# Autodesk Inventor assembly: shoot
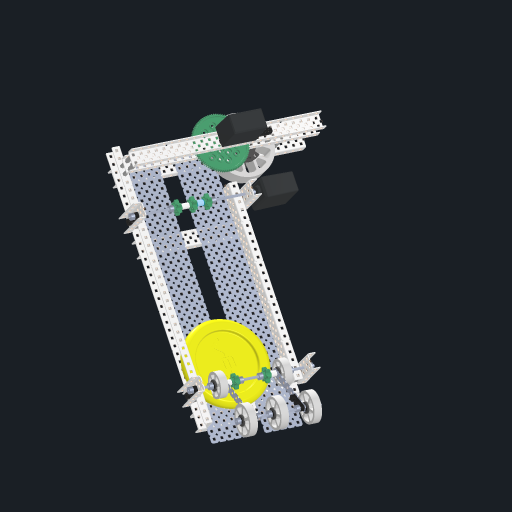
[picture p0: Inventor's stored thumbnail of the model, 512x512]
Saved by Autodesk Inventor 2023 (Build 270158000, 158)
## iProperties
Created: 2023-03-08
Part Number: shoot
Document SubType Name: Assembly
Designer: Windows Macbook
Author: Windows Macbook
## Documents named in this file (39)
- C:\Users\Windows Macbook\Desktop\VRC-SPIN-UP\Inventor\Assembly\Pre Worlds\V1\shoot.iam
- C:\Users\Windows Macbook\Desktop\VRC-SPIN-UP\Inventor\Structure\C Channel\Aluminum 1x2x1\Alu C 1x2x1x35.ipt
- C:\Users\Windows Macbook\Desktop\VRC-SPIN-UP\Inventor\Structure\C Channel\Aluminum 1x2x1\Alu C 1x2x1x14.ipt
- C:\Users\Windows Macbook\Desktop\VRC-SPIN-UP\Inventor\Structure\Plate\Steel\Steel Plate 5x25.ipt
- C:\Users\Windows Macbook\Desktop\VRC-SPIN-UP\Inventor\Structure\Plate\Steel\Steel Plate 5x10.ipt
- C:\Users\Windows Macbook\Desktop\VRC-SPIN-UP\Inventor\Structure\C Channel\Aluminum 1x2x1\Alu C 1x2x1x25.ipt
- C:\Users\Windows Macbook\Desktop\VRC-SPIN-UP\Inventor\Motion\Wheels\Flex Wheels\4 Flex, LS.iam
- C:\Users\Windows Macbook\Desktop\VRC-SPIN-UP\Inventor\Structure\Standoff\Standoff .50.ipt
- C:\Users\Windows Macbook\Desktop\VRC-SPIN-UP\Inventor\Structure\Standoff.ipt
- C:\Users\Windows Macbook\Desktop\VRC-SPIN-UP\Inventor\Structure\C Channel\Aluminum 1x3x1\Alu C 1x3x1x14.ipt
- C:\Users\Windows Macbook\Desktop\VRC-SPIN-UP\Inventor\Motion\Spacers\Spacer Nylon .375 OD\NSpacer .375 OD x .500.ipt
- C:\Users\Windows Macbook\Desktop\VRC-SPIN-UP\Inventor\Motion\Spacers\Spacer Nylon .375 OD.ipt
- C:\Users\Windows Macbook\Desktop\VRC-SPIN-UP\Inventor\Motion\Spacers\Spacer Nylon .375 OD\NSpacer .375 OD x .250.ipt
- C:\Users\Windows Macbook\Desktop\VRC-SPIN-UP\Inventor\Structure\Hardware\Screw Steel - Star.ipt
- C:\Users\Windows Macbook\Desktop\VRC-SPIN-UP\Inventor\Structure\Hardware\Screw Steel - Star\SScrew Star Smooth 1.000.ipt
- C:\Users\Windows Macbook\Desktop\VRC-SPIN-UP\Inventor\Structure\Hardware\Nut Nylock.ipt
- C:\Users\Windows Macbook\Desktop\VRC-SPIN-UP\Inventor\Motion\Shaft LS\Bearing Flat.ipt
- C:\Users\Windows Macbook\Desktop\VRC-SPIN-UP\Inventor\Motion\Spacers\Spacer Nylon .313 OD.ipt
- C:\Users\Windows Macbook\Desktop\VRC-SPIN-UP\Inventor\Motion\Gears\HS Gear\HS 12T Gear, Square.iam
- C:\Users\Windows Macbook\Desktop\VRC-SPIN-UP\Inventor\Motion\Gears\HS Gear.iam
- C:\Users\Windows Macbook\Desktop\VRC-SPIN-UP\Inventor\Motion\Gears\LS 84T Gear.ipt
- C:\Users\Windows Macbook\Desktop\VRC-SPIN-UP\Inventor\Motion\Spacers\Spacer Nylon .313 OD\NSpacer .313 OD x .125.ipt
- C:\Users\Windows Macbook\Desktop\VRC-SPIN-UP\Inventor\Motion\Spacers\Spacer Nylon .313 OD\NSpacer .313 OD x .250.ipt
- C:\Users\Windows Macbook\Desktop\VRC-SPIN-UP\Inventor\Structure\Standoff\Standoff 1.00.ipt
- C:\Users\Windows Macbook\Desktop\VRC-SPIN-UP\Inventor\Structure\Plate\Steel\Steel Plate 1x8.ipt
- C:\Users\Windows Macbook\Desktop\VRC-SPIN-UP\Inventor\Disk.ipt
- C:\Users\Windows Macbook\Desktop\VRC-SPIN-UP\Inventor\Structure\C Channel\Aluminum 1x2x1\Alu C 1x2x1x5.ipt
- C:\Users\Windows Macbook\Desktop\VRC-SPIN-UP\Inventor\Motion\Shaft LS\Shaft LS\Shaft LS 8.0.ipt
- C:\Users\Windows Macbook\Desktop\VRC-SPIN-UP\Inventor\Motion\Shaft LS\Shaft LS.ipt
- C:\Users\Windows Macbook\Desktop\VRC-SPIN-UP\Inventor\Motion\Wheels\Flex Wheels\1.625 Flex, LS.iam
- C:\Users\Windows Macbook\Desktop\VRC-SPIN-UP\Inventor\Motion\Reference Files\Shaft Collar Metal.ipt
- C:\Users\Windows Macbook\Desktop\VRC-SPIN-UP\Inventor\Motion\Wheels\Flex Wheels\2 Flex, LS.iam
- C:\Users\Windows Macbook\Desktop\VRC-SPIN-UP\Inventor\Motion\Shaft LS\Shaft LS\Shaft LS 5.5.ipt
- C:\Users\Windows Macbook\Desktop\VRC-SPIN-UP\Inventor\Motion\Sprockets\9P Sprocket.iam
- C:\Users\Windows Macbook\Desktop\VRC-SPIN-UP\Inventor\Motion\Spacers\Spacer Nylon .313 OD\NSpacer .313 OD x .375.ipt
- C:\Users\Windows Macbook\Desktop\VRC-SPIN-UP\Inventor\Motion\Sprockets\9P Sprocket\9P 6T Sprocket, Square.iam
- C:\Users\Windows Macbook\Desktop\VRC-SPIN-UP\Inventor\Electronics\V5 Simple Motor.ipt
- C:\Users\Windows Macbook\Desktop\VRC-SPIN-UP\Inventor\Structure\Standoff\Standoff .75.ipt
- C:\Users\Windows Macbook\Desktop\VRC-SPIN-UP\Inventor\Motion\Spacers\Spacer Nylon .313 OD\NSpacer .313 OD x .500.ipt
## Components (97 placed, 31 different names)
1. Alu C 1x2x1x35:1 — Insert:1, Insert:2, Insert:15, Insert:16, Insert:18, Insert:19, Insert:22, Insert:23, Insert:43, Insert:44, Insert:91, Insert:92
2. Alu C 1x2x1x25:1 — Insert:17, Insert:117, Insert:118, Insert:119, Insert:120
3. Alu C 1x2x1x14:2 — Insert:1, Insert:2, Insert:7, Insert:8, Insert:9, Insert:10, Insert:24, Insert:26
4. Alu C 1x2x1x25:3 — Insert:5, Insert:6, Insert:69, Insert:70, Angle:1, Insert:96, Insert:97
5. Steel Plate 5x25:1 — Insert:9, Insert:10, Mate:1
6. Steel Plate 5x25:2 — Insert:7, Insert:8
7. Steel Plate 5x10:1
8. Steel Plate 5x10:2
9. Alu C 1x2x1x14:3 — Insert:15, Insert:16
10. 4 Flex, LS:1 [sub-assembly] — Insert:17, Insert:114
11. Standoff .75:1 — Insert:19, Insert:21
12. Standoff .75:2 — Insert:18, Insert:20
13. Alu C 1x2x1x25:2 — Insert:20, Insert:21, Insert:28, Insert:29, Insert:32, Insert:33, Insert:37, Insert:38, Insert:123, Insert:124
14. Alu C 1x3x1x14:1 — Insert:22, Insert:23, Insert:5, Insert:6
15. NSpacer .375 OD x .500:1 — Insert:24, Insert:25
16. NSpacer .375 OD x .250:2 — Insert:25, Insert:27
17. SScrew Star Smooth 1.000:1 — Insert:26
18. Nut Nylock:1 — Insert:27
19. Bearing Flat:1 — Insert:28, Insert:29, Insert:30
20. NSpacer .313 OD x .250:1 — Insert:30, Insert:31
21. HS 12T Gear, Square:1 [sub-assembly] — Insert:31
22. LS 84T Gear:1 — Insert:34, Insert:36
23. Bearing Flat:2 — Insert:32, Insert:33, Insert:35
24. NSpacer .313 OD x .125:2 — Insert:34, Insert:35
25. NSpacer .313 OD x .125:3 — Insert:36
26. Standoff 1.00:3 — Insert:38
27. Standoff 1.00:4 — Insert:37
28. Alu C 1x2x1x25:4 — Insert:121, Insert:122, Insert:125, Insert:126, Insert:128, Insert:129
29. Steel Plate 1x8:1 — Insert:52, Insert:53, Insert:54, Insert:56, Insert:78
30. Alu C 1x2x1x5:2 — Insert:45, Insert:46, Insert:47, Insert:48, Insert:49
31. Standoff .50:7 — Insert:44, Insert:46
32. Standoff .50:8 — Insert:43, Insert:45
33. Disk:2 — Mate:1
34. Bearing Flat:3 — Insert:47, Insert:48, Flush:1, Cylindrical:1, Insert:104
35. Shaft LS 8.0:1 — Flush:1, Cylindrical:1
36. 1.625 Flex, LS:1 [sub-assembly] — Insert:49, Insert:50, Insert:56
37. Shaft Collar Metal:1 — Insert:50
38. 2 Flex, LS:1 [sub-assembly] — Insert:52, Insert:58
39. Shaft Collar Metal:2 — Insert:55, Insert:76
40. Bearing Flat:4 — Insert:53, Insert:54, Insert:55
41. NSpacer .313 OD x .375:5 — Insert:78, Insert:79
42. Shaft Collar Metal:4 — Insert:58, Flush:2, Cylindrical:2
43. Steel Plate 1x8:2 — Insert:77
44. 1.625 Flex, LS:2 [sub-assembly] — Insert:72, Insert:73
45. 2 Flex, LS:2 [sub-assembly] — Insert:66
46. Shaft Collar Metal:6
47. Bearing Flat:5
48. NSpacer .313 OD x .375:4 — Insert:77, Insert:80
49. Shaft Collar Metal:8 — Insert:66, Cylindrical:3
50. Alu C 1x2x1x5:3 — Insert:71, Angle:1, Insert:72
51. Bearing Flat:6 — Insert:103
52. Standoff .50:9 — Insert:69
53. Standoff .50:10 — Insert:70, Insert:71
54. Shaft Collar Metal:9 — Insert:73
55. Shaft LS 5.5:2 — Flush:2, Cylindrical:2, Cylindrical:3
56. 2 Flex, LS:3 [sub-assembly] — Insert:74, Insert:75
57. Shaft Collar Metal:10 — Insert:75
58. Shaft Collar Metal:11 — Insert:74, Insert:76
59. 9P 6T Sprocket, Square:1 [sub-assembly] — Insert:79, Insert:82
60. 9P 6T Sprocket, Square:2 [sub-assembly] — Insert:80, Insert:81
61. Shaft Collar Metal:12 — Insert:82
62. Shaft Collar Metal:13 — Insert:81
63. Alu C 1x2x1x5:4 — Insert:95
64. Standoff .50:11 — Insert:92
65. Standoff .50:12 — Insert:91
66. Bearing Flat:7 — Insert:101
67. Shaft LS 8.0:3
68. Alu C 1x2x1x5:5 — Insert:90, Insert:100
69. Bearing Flat:8 — Insert:105, Insert:106, Insert:110
70. Standoff .50:13 — Insert:90, Insert:97
71. Standoff .50:14 — Insert:96
72. 9P 6T Sprocket, Square:3 [sub-assembly] — Insert:94, Insert:139
73. Shaft Collar Metal:15 — Insert:94, Insert:95
74. 9P 6T Sprocket, Square:4 [sub-assembly] — Insert:140
75. Shaft Collar Metal:16 — Insert:100
76. Shaft Collar Metal:19 — Insert:103
77. Shaft Collar Metal:20 — Insert:101
78. Shaft Collar Metal:21 — Insert:104
79. V5 Simple Motor:1 — Insert:105, Insert:106
80. V5 Simple Motor:2 — Insert:130, Insert:131
81. Shaft Collar Metal:23 — Insert:110
82. Shaft Collar Metal:24 — Insert:113
83. Shaft Collar Metal:26 — Insert:111
84. NSpacer .313 OD x .250:6 — Insert:114
85. Standoff 1.00:15 — Insert:115
86. Standoff .75:16 — Insert:115, Insert:118
87. Standoff 1.00:17
88. Standoff .75:18 — Insert:117
89. Bearing Flat:9 — Insert:119, Insert:120, Insert:113
90. Bearing Flat:10 — Insert:121, Insert:111, Insert:122, Insert:130, Insert:131
91. Standoff 1.00:19 — Insert:123, Insert:126
92. Standoff 1.00:20 — Insert:124, Insert:125
93. Shaft Collar Metal:27
94. Bearing Flat:11 — Insert:128, Insert:129
95. 9P 6T Sprocket, Square:5 [sub-assembly] — Insert:141
96. NSpacer .313 OD x .500:8 — Insert:139, Insert:141
97. NSpacer .313 OD x .500:9 — Insert:140
## Relationships (128: Insert 119, CylindricalJoint 4, Flush 3, Mate 1, Angle 1)
- Insert:1: Alu C 1x2x1x35:1 ↔ Alu C 1x2x1x14:2
- Insert:2: Alu C 1x2x1x35:1 ↔ Alu C 1x2x1x14:2
- [Insert]: Alu C 1x2x1x35:1 ↔ Alu C 1x2x1x25:1
- [Insert]: Alu C 1x2x1x35:1 ↔ Alu C 1x2x1x25:1
- Insert:5: Alu C 1x2x1x25:3 ↔ Alu C 1x3x1x14:1
- Insert:6: Alu C 1x2x1x25:3 ↔ Alu C 1x3x1x14:1
- Insert:7: Alu C 1x2x1x14:2 ↔ Steel Plate 5x25:2
- Insert:8: Alu C 1x2x1x14:2 ↔ Steel Plate 5x25:2
- Insert:9: Alu C 1x2x1x14:2 ↔ Steel Plate 5x25:1
- Insert:10: Alu C 1x2x1x14:2 ↔ Steel Plate 5x25:1
- [Insert]: Alu C 1x2x1x25:1 ↔ Steel Plate 5x10:1
- [Insert]: Alu C 1x2x1x25:1 ↔ Steel Plate 5x10:1
- [Insert]: Alu C 1x2x1x25:1 ↔ Steel Plate 5x10:2
- [Insert]: Alu C 1x2x1x25:1 ↔ Steel Plate 5x10:2
- Insert:15: Alu C 1x2x1x35:1 ↔ Alu C 1x2x1x14:3
- Insert:16: Alu C 1x2x1x35:1 ↔ Alu C 1x2x1x14:3
- Insert:17: Alu C 1x2x1x25:1 ↔ 4 Flex, LS:1
- Insert:18: Alu C 1x2x1x35:1 ↔ Standoff .75:2
- Insert:19: Alu C 1x2x1x35:1 ↔ Standoff .75:1
- Insert:20: Standoff .75:2 ↔ Alu C 1x2x1x25:2
- Insert:21: Standoff .75:1 ↔ Alu C 1x2x1x25:2
- Insert:22: Alu C 1x2x1x35:1 ↔ Alu C 1x3x1x14:1
- Insert:23: Alu C 1x2x1x35:1 ↔ Alu C 1x3x1x14:1
- Insert:24: Alu C 1x2x1x14:2 ↔ NSpacer .375 OD x .500:1
- Insert:25: NSpacer .375 OD x .500:1 ↔ NSpacer .375 OD x .250:2
- Insert:26: Alu C 1x2x1x14:2 ↔ SScrew Star Smooth 1.000:1
- Insert:27: NSpacer .375 OD x .250:2 ↔ Nut Nylock:1
- Insert:28: Alu C 1x2x1x25:2 ↔ Bearing Flat:1
- Insert:29: Alu C 1x2x1x25:2 ↔ Bearing Flat:1
- Insert:30: Bearing Flat:1 ↔ NSpacer .313 OD x .250:1
- Insert:31: NSpacer .313 OD x .250:1 ↔ HS 12T Gear, Square:1
- Insert:32: Alu C 1x2x1x25:2 ↔ Bearing Flat:2
- Insert:33: Alu C 1x2x1x25:2 ↔ Bearing Flat:2
- Insert:34: LS 84T Gear:1 ↔ NSpacer .313 OD x .125:2
- Insert:35: Bearing Flat:2 ↔ NSpacer .313 OD x .125:2
- Insert:36: LS 84T Gear:1 ↔ NSpacer .313 OD x .125:3
- Insert:37: Alu C 1x2x1x25:2 ↔ Standoff 1.00:4
- Insert:38: Alu C 1x2x1x25:2 ↔ Standoff 1.00:3
- Insert:43: Alu C 1x2x1x35:1 ↔ Standoff .50:8
- Insert:44: Alu C 1x2x1x35:1 ↔ Standoff .50:7
- Insert:45: Alu C 1x2x1x5:2 ↔ Standoff .50:8
- Insert:46: Alu C 1x2x1x5:2 ↔ Standoff .50:7
- Mate:1: Steel Plate 5x25:1 ↔ Disk:2
- Insert:47: Alu C 1x2x1x5:2 ↔ Bearing Flat:3
- Insert:48: Alu C 1x2x1x5:2 ↔ Bearing Flat:3
- Flush:1: Bearing Flat:3 ↔ Shaft LS 8.0:1
- Cylindrical:1: Bearing Flat:3 ↔ Shaft LS 8.0:1
- Insert:49 (25.4 mm): Alu C 1x2x1x5:2 ↔ 1.625 Flex, LS:1
- Insert:50: 1.625 Flex, LS:1 ↔ Shaft Collar Metal:1
- Insert:52: Steel Plate 1x8:1 ↔ 2 Flex, LS:1
- Insert:53: Steel Plate 1x8:1 ↔ Bearing Flat:4
- Insert:54: Steel Plate 1x8:1 ↔ Bearing Flat:4
- Insert:55: Shaft Collar Metal:2 ↔ Bearing Flat:4
- Insert:56: Steel Plate 1x8:1 ↔ 1.625 Flex, LS:1
- Insert:58: 2 Flex, LS:1 ↔ Shaft Collar Metal:4
- [Insert]: Steel Plate 1x8:2 ↔ 2 Flex, LS:2
- [Insert]: Steel Plate 1x8:2 ↔ Bearing Flat:5
- [Insert]: Steel Plate 1x8:2 ↔ Bearing Flat:5
- [Insert]: Shaft Collar Metal:6 ↔ Bearing Flat:5
- [Insert]: Steel Plate 1x8:2 ↔ 1.625 Flex, LS:2
- Insert:66: 2 Flex, LS:2 ↔ Shaft Collar Metal:8
- [Insert]: Alu C 1x2x1x5:3 ↔ Bearing Flat:6
- [Insert]: Alu C 1x2x1x5:3 ↔ Bearing Flat:6
- Insert:69: Alu C 1x2x1x25:3 ↔ Standoff .50:9
- Insert:70: Alu C 1x2x1x25:3 ↔ Standoff .50:10
- Insert:71: Alu C 1x2x1x5:3 ↔ Standoff .50:10
- Angle:1 (0 deg): Alu C 1x2x1x25:3 ↔ Alu C 1x2x1x5:3
- Insert:72 (25.4 mm): 1.625 Flex, LS:2 ↔ Alu C 1x2x1x5:3
- Insert:73: 1.625 Flex, LS:2 ↔ Shaft Collar Metal:9
- Flush:2: Shaft Collar Metal:4 ↔ Shaft LS 5.5:2
- Cylindrical:2: Shaft Collar Metal:4 ↔ Shaft LS 5.5:2
- Cylindrical:3: Shaft Collar Metal:8 ↔ Shaft LS 5.5:2
- Insert:74: 2 Flex, LS:3 ↔ Shaft Collar Metal:11
- Insert:75: 2 Flex, LS:3 ↔ Shaft Collar Metal:10
- Insert:76 (12.7 mm): Shaft Collar Metal:2 ↔ Shaft Collar Metal:11
- Insert:77: Steel Plate 1x8:2 ↔ NSpacer .313 OD x .375:4
- Insert:78: Steel Plate 1x8:1 ↔ NSpacer .313 OD x .375:5
- Insert:79: NSpacer .313 OD x .375:5 ↔ 9P 6T Sprocket, Square:1
- Insert:80: NSpacer .313 OD x .375:4 ↔ 9P 6T Sprocket, Square:2
- Insert:81: 9P 6T Sprocket, Square:2 ↔ Shaft Collar Metal:13
- Insert:82: 9P 6T Sprocket, Square:1 ↔ Shaft Collar Metal:12
- [Insert]: Alu C 1x2x1x5:4 ↔ Standoff .50:12
- [Insert]: Alu C 1x2x1x5:4 ↔ Standoff .50:11
- [Insert]: Alu C 1x2x1x5:4 ↔ Bearing Flat:7
- [Insert]: Alu C 1x2x1x5:4 ↔ Bearing Flat:7
- [Flush]: Bearing Flat:7 ↔ Shaft LS 8.0:3
- [CylindricalJoint]: Bearing Flat:7 ↔ Shaft LS 8.0:3
- [Insert]: Alu C 1x2x1x5:5 ↔ Bearing Flat:8
- [Insert]: Alu C 1x2x1x5:5 ↔ Bearing Flat:8
- [Insert]: Alu C 1x2x1x5:5 ↔ Standoff .50:14
- Insert:90: Alu C 1x2x1x5:5 ↔ Standoff .50:13
- Insert:91: Alu C 1x2x1x35:1 ↔ Standoff .50:12
- Insert:92: Alu C 1x2x1x35:1 ↔ Standoff .50:11
- Insert:94: 9P 6T Sprocket, Square:3 ↔ Shaft Collar Metal:15
- Insert:95 (50.8 mm): Alu C 1x2x1x5:4 ↔ Shaft Collar Metal:15
- Insert:96: Alu C 1x2x1x25:3 ↔ Standoff .50:14
- Insert:97: Alu C 1x2x1x25:3 ↔ Standoff .50:13
- [Insert]: 9P 6T Sprocket, Square:4 ↔ Shaft Collar Metal:16
- Insert:100 (50.8 mm): Alu C 1x2x1x5:5 ↔ Shaft Collar Metal:16
- Insert:101: Bearing Flat:7 ↔ Shaft Collar Metal:20
- Insert:103: Bearing Flat:6 ↔ Shaft Collar Metal:19
- Insert:104: Bearing Flat:3 ↔ Shaft Collar Metal:21
- Insert:105: Bearing Flat:8 ↔ V5 Simple Motor:1
- Insert:106: Bearing Flat:8 ↔ V5 Simple Motor:1
- Insert:110: Bearing Flat:8 ↔ Shaft Collar Metal:23
- Insert:111: Shaft Collar Metal:26 ↔ Bearing Flat:10
- Insert:113: Shaft Collar Metal:24 ↔ Bearing Flat:9
- Insert:114: 4 Flex, LS:1 ↔ NSpacer .313 OD x .250:6
- Insert:115: Standoff 1.00:15 ↔ Standoff .75:16
- [Insert]: Standoff 1.00:17 ↔ Standoff .75:18
- Insert:117: Alu C 1x2x1x25:1 ↔ Standoff .75:18
- Insert:118: Alu C 1x2x1x25:1 ↔ Standoff .75:16
- Insert:119: Alu C 1x2x1x25:1 ↔ Bearing Flat:9
- Insert:120: Alu C 1x2x1x25:1 ↔ Bearing Flat:9
- Insert:121: Alu C 1x2x1x25:4 ↔ Bearing Flat:10
- Insert:122: Alu C 1x2x1x25:4 ↔ Bearing Flat:10
- Insert:123: Alu C 1x2x1x25:2 ↔ Standoff 1.00:19
- Insert:124: Alu C 1x2x1x25:2 ↔ Standoff 1.00:20
- Insert:125: Alu C 1x2x1x25:4 ↔ Standoff 1.00:20
- Insert:126: Alu C 1x2x1x25:4 ↔ Standoff 1.00:19
- [Insert]: Shaft Collar Metal:27 ↔ Bearing Flat:11
- Insert:128: Alu C 1x2x1x25:4 ↔ Bearing Flat:11
- Insert:129: Alu C 1x2x1x25:4 ↔ Bearing Flat:11
- Insert:130: V5 Simple Motor:2 ↔ Bearing Flat:10
- Insert:131: V5 Simple Motor:2 ↔ Bearing Flat:10
- Insert:139: 9P 6T Sprocket, Square:3 ↔ NSpacer .313 OD x .500:8
- Insert:140: 9P 6T Sprocket, Square:4 ↔ NSpacer .313 OD x .500:9
- Insert:141: 9P 6T Sprocket, Square:5 ↔ NSpacer .313 OD x .500:8
## Named parameters: d65_d57 = 0 mm, d66_d58 = 0 mm, d67_d59 = 0 mm, d68_d60 = 0 mm, d69_d61 = 0 mm, d72_d49 = 0 mm, d73_d50 = 0 mm, d95_d46 = 0 mm, d96_d47 = 0 mm, d97_d49 = 0 mm, d98_d50 = 0 mm, d99_d51 = 0 mm, d100_d52 = 141.796211 deg, d101_d77 = 0 mm, d102_d53 = 0 mm, d103_d72_d49 = 0 mm, d104_d73_d50 = 0 mm, d113_d108_d94 = 0 mm, d131_d130 = 0 mm, d142_d126 = 0 mm
